# Autodesk Inventor assembly: Vitme
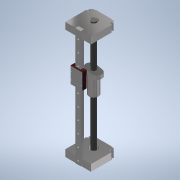
[picture p0: Inventor's stored thumbnail of the model, 180x180]
Saved by Autodesk Inventor 2021.3 (Build 253353000, 353)
## iProperties
Created: 2021-06-01
Part Number: Vitme
Document SubType Name: Assembly
Designer: vivek
Author: vivek
## Documents named in this file (6)
- C:\Users\vivek\OneDrive\Documents\II Sem\EE\Pattern Drawing Bot\Final3DModel\Rod_Set.iam
- C:\Users\vivek\OneDrive\Documents\II Sem\EE\Pattern Drawing Bot\Final3DModel\Holder.ipt
- C:\Users\vivek\OneDrive\Documents\II Sem\EE\Pattern Drawing Bot\Final3DModel\Rotator.ipt
- C:\Users\vivek\OneDrive\Documents\II Sem\EE\Pattern Drawing Bot\Final3DModel\Pen_Holder.ipt
- C:\Users\vivek\OneDrive\Documents\II Sem\EE\Pattern Drawing Bot\Final3DModel\Stand.ipt
- C:\Users\vivek\OneDrive\Documents\II Sem\EE\Pattern Drawing Bot\Final3DModel\Rod.ipt
## Components (6 placed, 5 different names)
1. Holder:1 — Mate:2, Flush:1, Mate:9
2. Rotator:1 — Mate:1
3. Pen_Holder:1 — Mate:7, Mate:8
4. Stand:1 — Mate:5, Flush:3, Mate:6, Mate:7, Mate:8, Mate:9
5. Rod:1 — Mate:1, Mate:2, Flush:1, Mate:4, Flush:2
6. Holder:2 — Mate:4, Flush:2, Mate:5, Flush:3, Mate:6
## Relationships (11: Mate 8, Flush 3)
- Mate:1: Rotator:1 ↔ Rod:1
- Mate:2: Holder:1 ↔ Rod:1
- Flush:1: Holder:1 ↔ Rod:1
- Mate:4: Rod:1 ↔ Holder:2
- Flush:2: Rod:1 ↔ Holder:2
- Mate:5: Stand:1 ↔ Holder:2
- Flush:3: Stand:1 ↔ Holder:2
- Mate:6: Stand:1 ↔ Holder:2
- Mate:7: Pen_Holder:1 ↔ Stand:1
- Mate:8: Pen_Holder:1 ↔ Stand:1
- Mate:9: Holder:1 ↔ Stand:1
